# Autodesk Inventor assembly: 2013 Drive in a Day with wheels
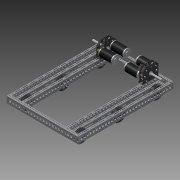
[picture p0: Inventor's stored thumbnail of the model, 180x180]
Saved by Autodesk Inventor 2013 (Build 170138000, 138)
## iProperties
Created: 2013-05-24
Part Number: 2013 Drive in a Day with wheels
Document SubType Name: Assembly
Designer: natsidhu
Author: natsidhu
## Documents named in this file (5)
- \\lmss\STUDENTS\Robotics\CAD Files\COTS Parts\Kit Frame - VexPro\2013 Drive in a Day with wheels.iam
- \\lmss\STUDENTS\Robotics\CAD Files\COTS Parts\Kit Frame - VexPro\2013 Drive in a Day Frame.iam
- \\lmss\STUDENTS\Robotics\CAD Files\COTS Parts\Kit Frame - VexPro\drive in a day axile tube.ipt
- \\lmss\STUDENTS\Robotics\CAD Files\COTS Parts\Kit Frame - VexPro\Wheel 42T and 34T drive in a day.iam
- \\lmss\STUDENTS\Robotics\CAD Files\COTS Parts\Gearboxes\VexPro 64 Single Stage Gearbox.iam
## Components (15 placed, 4 different names)
1. 2013 Drive in a Day Frame:1 [sub-assembly] — Mate:1, Mate:2, Mate:7, Mate:8, Mate:10, Mate:11, Mate:12, Mate:13, Mate:18, Mate:19, Mate:20, Mate:21, Flush:5, Mate:24, Mate:25, Flush:6, Mate:26
2. drive in a day axile tube:2 — Mate:10, Mate:11, Mate:15
3. drive in a day axile tube:5 — Mate:7, Mate:8, Mate:16
4. drive in a day axile tube:6 — Mate:1, Mate:2, Mate:17
5. drive in a day axile tube:7 — Mate:12, Mate:13, Mate:14
6. drive in a day axile tube:8 — Mate:20, Mate:21, Mate:22
7. drive in a day axile tube:9 — Mate:18, Mate:19, Mate:23
8. Wheel 42T and 34T drive in a day:1 [sub-assembly] — Flush:1, Mate:17
9. Wheel 42T and 34T drive in a day:2 [sub-assembly] — Mate:14, Flush:2, Flush:4
10. Wheel 42T and 34T drive in a day:3 [sub-assembly] — Mate:16, Flush:1, Flush:3
11. Wheel 42T and 34T drive in a day:4 [sub-assembly] — Mate:15, Flush:2
12. Wheel 42T and 34T drive in a day:5 [sub-assembly] — Flush:4, Mate:23
13. Wheel 42T and 34T drive in a day:6 [sub-assembly] — Flush:3, Mate:22
14. VexPro 64 Single Stage Gearbox:1 [sub-assembly] — Flush:5, Mate:26
15. VexPro 64 Single Stage Gearbox:2 [sub-assembly] — Mate:24, Mate:25, Flush:6
## Relationships (27: Mate 21, Flush 6)
- Mate:1: 2013 Drive in a Day Frame:1 ↔ drive in a day axile tube:6
- Mate:2: 2013 Drive in a Day Frame:1 ↔ drive in a day axile tube:6
- Mate:7: 2013 Drive in a Day Frame:1 ↔ drive in a day axile tube:5
- Mate:8: 2013 Drive in a Day Frame:1 ↔ drive in a day axile tube:5
- Mate:10: 2013 Drive in a Day Frame:1 ↔ drive in a day axile tube:2
- Mate:11: 2013 Drive in a Day Frame:1 ↔ drive in a day axile tube:2
- Mate:12: 2013 Drive in a Day Frame:1 ↔ drive in a day axile tube:7
- Mate:13: 2013 Drive in a Day Frame:1 ↔ drive in a day axile tube:7
- Mate:14: drive in a day axile tube:7 ↔ Wheel 42T and 34T drive in a day:2
- Mate:15: drive in a day axile tube:2 ↔ Wheel 42T and 34T drive in a day:4
- Mate:16: drive in a day axile tube:5 ↔ Wheel 42T and 34T drive in a day:3
- Flush:1: Wheel 42T and 34T drive in a day:1 ↔ Wheel 42T and 34T drive in a day:3
- Mate:17: drive in a day axile tube:6 ↔ Wheel 42T and 34T drive in a day:1
- Flush:2: Wheel 42T and 34T drive in a day:2 ↔ Wheel 42T and 34T drive in a day:4
- Mate:18: 2013 Drive in a Day Frame:1 ↔ drive in a day axile tube:9
- Mate:19: 2013 Drive in a Day Frame:1 ↔ drive in a day axile tube:9
- Mate:20: 2013 Drive in a Day Frame:1 ↔ drive in a day axile tube:8
- Mate:21: 2013 Drive in a Day Frame:1 ↔ drive in a day axile tube:8
- Flush:3: Wheel 42T and 34T drive in a day:3 ↔ Wheel 42T and 34T drive in a day:6
- Mate:22: drive in a day axile tube:8 ↔ Wheel 42T and 34T drive in a day:6
- Flush:4: Wheel 42T and 34T drive in a day:2 ↔ Wheel 42T and 34T drive in a day:5
- Mate:23: drive in a day axile tube:9 ↔ Wheel 42T and 34T drive in a day:5
- Flush:5: 2013 Drive in a Day Frame:1 ↔ VexPro 64 Single Stage Gearbox:1
- Mate:24: 2013 Drive in a Day Frame:1 ↔ VexPro 64 Single Stage Gearbox:2
- Mate:25: 2013 Drive in a Day Frame:1 ↔ VexPro 64 Single Stage Gearbox:2
- Flush:6: 2013 Drive in a Day Frame:1 ↔ VexPro 64 Single Stage Gearbox:2
- Mate:26: 2013 Drive in a Day Frame:1 ↔ VexPro 64 Single Stage Gearbox:1
